# Autodesk Inventor assembly: robot_assembly
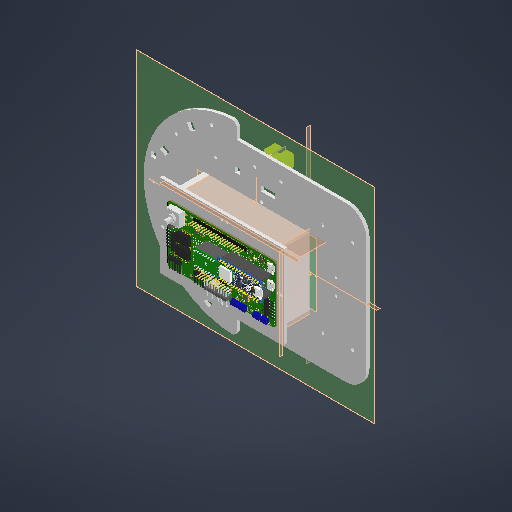
[picture p0: Inventor's stored thumbnail of the model, 512x512]
Saved by Autodesk Inventor 2026.1 (Build 301233020, 233B)
## iProperties
Created: 2025-10-09
Part Number: robot_assembly
Document SubType Name: Assembly
Designer: osama
Author: osama
## Documents named in this file (10)
- C:\Users\osama\OneDrive\Documents\Inventor\CAD_fwm509\robot_assembly.iam
- C:\Users\osama\OneDrive\Documents\Inventor\CAD_fwm509\ARB Board CAD model.ipt
- C:\Users\osama\OneDrive\Documents\Inventor\CAD_fwm509\base_plate.ipt
- C:\Users\osama\OneDrive\Documents\Inventor\CAD_fwm509\MotorHolder.ipt
- C:\Users\osama\OneDrive\Documents\Inventor\CAD_fwm509\MotorHolder_MIR1.ipt
- C:\Users\osama\OneDrive\Documents\Inventor\CAD_fwm509\0.75in Ball Caster (Pololu).ipt
- C:\Users\osama\OneDrive\Documents\Inventor\CAD_fwm509\0.75in Ball Caster (Pololu)_MIR.ipt
- C:\Users\osama\OneDrive\Documents\Inventor\CAD_fwm509\top_plate.ipt
- C:\Users\osama\OneDrive\Documents\Inventor\CAD_fwm509\battery2.ipt
- C:\Users\osama\OneDrive\Documents\Inventor\CAD_fwm509\topplate_v2.ipt
## Components (9 placed, 9 different names)
1. ARB Board CAD model:1 — Mate:19
2. base_plate:1 — Flush:3, Mate:1, Mate:2, Mate:3, Mate:4, Mate:5, Mate:8, Mate:15, Mate:16, Mate:17
3. battery2:1 — Mate:15, Mate:16, Mate:17, Flush:10, Flush:14, Flush:15, Mate:18
4. top_plate:2
5. topplate_v2:1 — Flush:11, Flush:13, Flush:15, Mate:18, Mate:19
6. MotorHolder:2 — Flush:3, Mate:1, Mate:2
7. MotorHolder_MIR1:1
8. 0.75in Ball Caster (Pololu):1 — Mate:3, Mate:4
9. 0.75in Ball Caster (Pololu)_MIR:1 — Mate:8
## Component patterns: (2 elements, first: MotorHolder:2), (2 elements, first: 0.75in Ball Caster (Pololu):1)
## Relationships (18: Mate 11, Flush 7)
- Flush:3: base_plate:1 ↔ MotorHolder:2
- Mate:1 (30 mm): base_plate:1 ↔ MotorHolder:2
- Mate:2: base_plate:1 ↔ MotorHolder:2
- Mate:3: base_plate:1 ↔ 0.75in Ball Caster (Pololu):1
- Mate:4: base_plate:1 ↔ 0.75in Ball Caster (Pololu):1
- Mate:5: base_plate:1
- Mate:8: base_plate:1 ↔ 0.75in Ball Caster (Pololu)_MIR:1
- Mate:15 (55 mm): base_plate:1 ↔ battery2:1
- Mate:16: base_plate:1 ↔ battery2:1
- Mate:17 (32.5 mm): base_plate:1 ↔ battery2:1
- Flush:10: battery2:1
- Flush:11: topplate_v2:1
- Flush:12 (9 mm)
- Flush:13: topplate_v2:1
- Flush:14: battery2:1
- Flush:15 (-7.5 mm): battery2:1 ↔ topplate_v2:1
- Mate:18 (7 mm): battery2:1 ↔ topplate_v2:1
- Mate:19: ARB Board CAD model:1 ↔ topplate_v2:1
